# Autodesk Inventor assembly: Assembly1
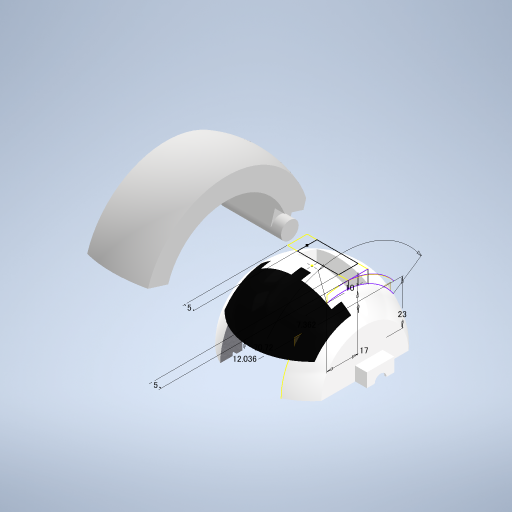
[picture p0: Inventor's stored thumbnail of the model, 512x512]
Saved by Autodesk Inventor 2023 (Build 270158000, 158)
## iProperties
Created: 2022-10-31
Part Number: Assembly1
Document SubType Name: Assembly
Designer: ellie
Author: ellie
## Documents named in this file (4)
- C:\Users\ellie\Documents\github\tanekonsat2022_runback\machinary\body\Assembly1.iam
- C:\Users\ellie\Documents\github\tanekonsat2022_runback\machinary\body\body back for main 3.ipt
- C:\Users\ellie\Documents\github\tanekonsat2022_runback\machinary\parts\tail trying like shit.ipt
- C:\Users\ellie\Documents\github\tanekonsat2022_runback\machinary\body\body back 2.ipt
## Components (3 placed, 2 different names)
1. body back:2 — メイト:1, メイト:2, メイト:3
2. tail trying like shit:1
3. body back:3 — メイト:1, メイト:2, メイト:3
## Relationships (3: Mate 3)
- メイト:1 [Mate]: body back:2 ↔ body back:3
- メイト:2 [Mate]: body back:2 ↔ body back:3
- メイト:3 [Mate]: body back:2 ↔ body back:3
